# Autodesk Inventor assembly: Tiger
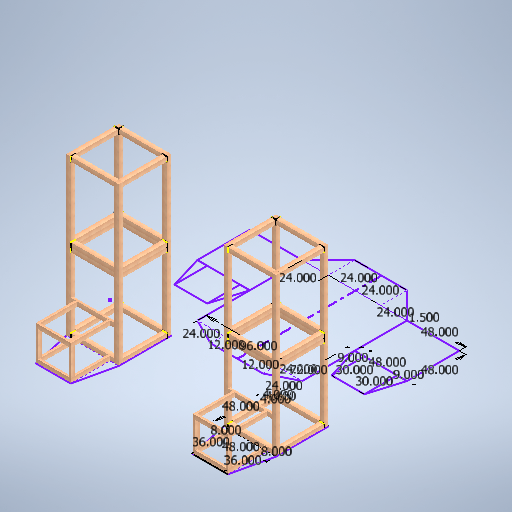
[picture p0: Inventor's stored thumbnail of the model, 512x512]
Saved by Autodesk Inventor 2025 (Build 290162000, 162)
## iProperties
Created: 2024-06-05
Part Number: Tiger
Document SubType Name: Assembly
Designer: Cupri
Mass: 180546 g
Surface Area: 136258 cm^2
Volume: 328266 cm^3
Density: 0.55 g/cm^3
Author: Cupri
## Documents named in this file (13)
- C:\Users\Cupri\OneDrive\Documents\TigerBurn\USCTigerBurn24\v1\Tiger.iam
- C:\Users\Cupri\OneDrive\Documents\TigerBurn\USCTigerBurn24\Standard Timber\4x4x72.ipt
- C:\Users\Cupri\OneDrive\Documents\TigerBurn\USCTigerBurn24\Standard Timber\4x4x40.ipt
- C:\Users\Cupri\OneDrive\Documents\TigerBurn\USCTigerBurn24\Standard Timber\2x4x36.ipt
- C:\Users\Cupri\OneDrive\Documents\TigerBurn\USCTigerBurn24\Standard Timber\2x4x40.ipt
- C:\Users\Cupri\OneDrive\Documents\TigerBurn\USCTigerBurn24\Standard Timber\2x4x24.ipt
- C:\Users\Cupri\OneDrive\Documents\TigerBurn\USCTigerBurn24\Standard Timber\2x4x28.ipt
- C:\Users\Cupri\OneDrive\Documents\TigerBurn\USCTigerBurn24\v1\Tiger\AIP\FEA\epzzwi8io.fins
- C:\Users\Cupri\OneDrive\Documents\TigerBurn\USCTigerBurn24\v1\Tiger\AIP\FEA\epzzwi8io.fsat
- C:\Users\Cupri\OneDrive\Documents\TigerBurn\USCTigerBurn24\v1\Tiger\AIP\FEA\epzzwi8io.ftes
- C:\Users\Cupri\OneDrive\Documents\TigerBurn\USCTigerBurn24\v1\Tiger\AIP\FEA\epzzwi8io.fwiz
- C:\Users\Cupri\OneDrive\Documents\TigerBurn\USCTigerBurn24\v1\Tiger\AIP\FEA\epzzwi8jk.fmsh
- C:\Users\Cupri\OneDrive\Documents\TigerBurn\USCTigerBurn24\v1\Tiger\AIP\FEA\epzzwi8jl.fres
## Components (66 placed, 6 different names)
1. 4x4x72:9
2. 4x4x72:10
3. 4x4x40:17 — Flush:14
4. 4x4x40:18
5. 4x4x40:19 — Mate:19, Mate:20
6. 4x4x40:20 — Flush:13, Mate:18
7. 4x4x40:21
8. 4x4x40:22
9. 4x4x40:23
10. 4x4x40:24
11. 4x4x72:11
12. 4x4x72:12 — Mate:21
13. 4x4x72:13
14. 4x4x72:14
15. 4x4x40:25
16. 4x4x40:26
17. 4x4x40:27
18. 4x4x40:28
19. 4x4x40:29
20. 4x4x40:30
21. 4x4x40:31
22. 4x4x40:32
23. 4x4x72:15
24. 4x4x72:16
25. 2x4x40:2 — Mate:21, Mate:23
26. 2x4x36:5 — Mate:20
27. 2x4x36:6 — Mate:23, Mate:24
28. 2x4x36:7 — Mate:22
29. 2x4x36:8 — Mate:19
30. 2x4x24:3
31. 2x4x24:4 — Mate:22
32. 2x4x28:3 — Mate:24
33. 2x4x28:4
34. 4x4x72:1 — Rigid:1, Rigid:3, Rigid:10, Rigid:11
35. 4x4x72:2 — Rigid:2, Rigid:4, Rigid:8
36. 4x4x40:1 — Rigid:1, Rigid:2, Flush:14
37. 4x4x40:2 — Rigid:3, Rigid:5, Flush:13, Mate:18
38. 4x4x40:3 — Rigid:6, Mate:5, Mate:6, Flush:4, Flush:5
39. 4x4x40:4 — Rigid:4, Rigid:7
40. 4x4x40:5 — Rigid:8
41. 4x4x40:6 — Rigid:9, Rigid:23
42. 4x4x40:7 — Rigid:11
43. 4x4x40:8 — Rigid:10
44. 4x4x72:3 — Rigid:5, Rigid:6, Rigid:9, Mate:4, Flush:3
45. 4x4x72:4 — Rigid:7, Mate:7
46. 4x4x72:5
47. 4x4x72:6
48. 4x4x40:9
49. 4x4x40:10
50. 4x4x40:11 — Rigid:23
51. 4x4x40:12
52. 4x4x40:13
53. 4x4x40:14
54. 4x4x40:15
55. 4x4x40:16
56. 4x4x72:7
57. 4x4x72:8
58. 2x4x40:1 — Mate:4, Flush:3, Mate:5, Mate:8, Flush:6, Mate:9, Flush:7
59. 2x4x36:1 — Mate:6, Flush:4, Rigid:24
60. 2x4x36:2 — Mate:8, Flush:6
61. 2x4x36:3 — Mate:9, Flush:7, Mate:10, Rigid:26
62. 2x4x36:4 — Mate:7, Flush:5, Mate:10, Rigid:25, Rigid:27
63. 2x4x24:1 — Rigid:24
64. 2x4x24:2 — Rigid:25
65. 2x4x28:1 — Rigid:26
66. 2x4x28:2 — Rigid:27
## Relationships (86: WeldJoint 54, Mate 20, Flush 12)
- Rigid:1 [WeldJoint]: 4x4x72:1 ↔ 4x4x40:1
- Rigid:2 [WeldJoint]: 4x4x72:2 ↔ 4x4x40:1
- Rigid:3 [WeldJoint]: 4x4x72:1 ↔ 4x4x40:2
- Rigid:4 [WeldJoint]: 4x4x72:2 ↔ 4x4x40:4
- Rigid:5 [WeldJoint]: 4x4x40:2 ↔ 4x4x72:3
- Rigid:6 [WeldJoint]: 4x4x40:3 ↔ 4x4x72:3
- Rigid:7 [WeldJoint]: 4x4x40:4 ↔ 4x4x72:4
- Rigid:8 [WeldJoint]: 4x4x72:2 ↔ 4x4x40:5
- Rigid:9 [WeldJoint]: 4x4x40:6 ↔ 4x4x72:3
- Rigid:10 [WeldJoint]: 4x4x72:1 ↔ 4x4x40:8
- Rigid:11 [WeldJoint]: 4x4x72:1 ↔ 4x4x40:7
- [WeldJoint]: 4x4x72:5 ↔ 4x4x40:9
- [WeldJoint]: 4x4x72:6 ↔ 4x4x40:9
- [WeldJoint]: 4x4x72:5 ↔ 4x4x40:10
- [WeldJoint]: 4x4x72:6 ↔ 4x4x40:12
- [WeldJoint]: 4x4x40:10 ↔ 4x4x72:7
- [WeldJoint]: 4x4x40:11 ↔ 4x4x72:7
- [WeldJoint]: 4x4x40:12 ↔ 4x4x72:8
- [WeldJoint]: 4x4x72:6 ↔ 4x4x40:13
- [WeldJoint]: 4x4x40:14 ↔ 4x4x72:7
- [WeldJoint]: 4x4x72:5 ↔ 4x4x40:16
- [WeldJoint]: 4x4x72:5 ↔ 4x4x40:15
- Rigid:23 [WeldJoint]: 4x4x40:6 ↔ 4x4x40:11
- Mate:4: 4x4x72:3 ↔ 2x4x40:1
- Flush:3: 4x4x72:3 ↔ 2x4x40:1
- Mate:5 (609.6 mm): 4x4x40:3 ↔ 2x4x40:1
- Mate:6 (101.6 mm): 4x4x40:3 ↔ 2x4x36:1
- Flush:4: 4x4x40:3 ↔ 2x4x36:1
- Mate:7 (101.6 mm): 4x4x72:4 ↔ 2x4x36:4
- Flush:5: 4x4x40:3 ↔ 2x4x36:4
- Mate:8 (101.6 mm): 2x4x40:1 ↔ 2x4x36:2
- Flush:6: 2x4x40:1 ↔ 2x4x36:2
- Mate:9: 2x4x40:1 ↔ 2x4x36:3
- Flush:7: 2x4x40:1 ↔ 2x4x36:3
- Mate:10: 2x4x36:3 ↔ 2x4x36:4
- Rigid:24 [WeldJoint]: 2x4x36:1 ↔ 2x4x24:1
- Rigid:25 [WeldJoint]: 2x4x36:4 ↔ 2x4x24:2
- Rigid:26 [WeldJoint]: 2x4x36:3 ↔ 2x4x28:1
- Rigid:27 [WeldJoint]: 2x4x36:4 ↔ 2x4x28:2
- [WeldJoint]: 4x4x72:9 ↔ 4x4x40:17
- [WeldJoint]: 4x4x72:10 ↔ 4x4x40:17
- [WeldJoint]: 4x4x72:9 ↔ 4x4x40:18
- [WeldJoint]: 4x4x72:10 ↔ 4x4x40:20
- [WeldJoint]: 4x4x40:18 ↔ 4x4x72:11
- [WeldJoint]: 4x4x40:19 ↔ 4x4x72:11
- [WeldJoint]: 4x4x40:20 ↔ 4x4x72:12
- [WeldJoint]: 4x4x72:10 ↔ 4x4x40:21
- [WeldJoint]: 4x4x40:22 ↔ 4x4x72:11
- [WeldJoint]: 4x4x72:9 ↔ 4x4x40:24
- [WeldJoint]: 4x4x72:9 ↔ 4x4x40:23
- [WeldJoint]: 4x4x72:13 ↔ 4x4x40:25
- [WeldJoint]: 4x4x72:14 ↔ 4x4x40:25
- [WeldJoint]: 4x4x72:13 ↔ 4x4x40:26
- [WeldJoint]: 4x4x72:14 ↔ 4x4x40:28
- [WeldJoint]: 4x4x40:26 ↔ 4x4x72:15
- [WeldJoint]: 4x4x40:27 ↔ 4x4x72:15
- [WeldJoint]: 4x4x40:28 ↔ 4x4x72:16
- [WeldJoint]: 4x4x72:14 ↔ 4x4x40:29
- [WeldJoint]: 4x4x40:30 ↔ 4x4x72:15
- [WeldJoint]: 4x4x72:13 ↔ 4x4x40:32
- [WeldJoint]: 4x4x72:13 ↔ 4x4x40:31
- [WeldJoint]: 4x4x40:22 ↔ 4x4x40:27
- [Mate]: 4x4x72:11 ↔ 2x4x40:2
- [Flush]: 4x4x72:11 ↔ 2x4x40:2
- [Mate] (609.6 mm): 4x4x40:19 ↔ 2x4x40:2
- [Mate] (101.6 mm): 4x4x40:19 ↔ 2x4x36:5
- [Flush]: 4x4x40:19 ↔ 2x4x36:5
- [Mate] (101.6 mm): 4x4x72:12 ↔ 2x4x36:8
- [Flush]: 4x4x40:19 ↔ 2x4x36:8
- [Flush]: 2x4x40:2 ↔ 2x4x36:6
- [Mate]: 2x4x40:2 ↔ 2x4x36:7
- [Flush]: 2x4x40:2 ↔ 2x4x36:7
- [Mate]: 2x4x36:7 ↔ 2x4x36:8
- [WeldJoint]: 2x4x36:5 ↔ 2x4x24:3
- [WeldJoint]: 2x4x36:8 ↔ 2x4x24:4
- [WeldJoint]: 2x4x36:7 ↔ 2x4x28:3
- [WeldJoint]: 2x4x36:8 ↔ 2x4x28:4
- Flush:13: 4x4x40:20 ↔ 4x4x40:2
- Mate:18 (2438.4 mm): 4x4x40:20 ↔ 4x4x40:2
- Flush:14: 4x4x40:17 ↔ 4x4x40:1
- Mate:19: 4x4x40:19 ↔ 2x4x36:8
- Mate:20: 4x4x40:19 ↔ 2x4x36:5
- Mate:21: 4x4x72:12 ↔ 2x4x40:2
- Mate:22: 2x4x36:7 ↔ 2x4x24:4
- Mate:23: 2x4x40:2 ↔ 2x4x36:6
- Mate:24: 2x4x36:6 ↔ 2x4x28:3
## Named parameters: d40_d29 = 0 mm, d41_d30 = 0 mm, d42_d31 = 0 mm, d43_d32 = 0 mm, d44_d33 = 0 mm, d45_d34 = 0 mm, d46_d35 = 0 mm, d47_d36 = 0 mm, d48_d37 = 0 mm, d49_d38 = 0 mm, d50_d39 = 0 mm, sa_0 = 22241.1, d81_d51 = 0 mm, d82_d31 = 0 mm, d83_d32 = 0 mm, d84_d33 = 0 mm, d85_d34 = 0 mm, d86_d35 = 0 mm, d87_d36 = 0 mm, d88_d37 = 0 mm, d89_d38 = 0 mm, d90_d39 = 0 mm, d91_d40_d29 = 0 mm, d92_d41_d30 = 0 mm, d93_d42_d31 = 0 mm, d94_d43_d32 = 0 mm, d95_d44_d33 = 0 mm, d96_d45_d34 = 0 mm, d97_d46_d35 = 0 mm, d98_d47_d36 = 0 mm, d99_d48_d37 = 0 mm, d100_d49_d38 = 0 mm, d101_d50_d39 = 0 mm, d102_d29 = 0 mm, d103_d30 = 0 mm, d104_d75 = 0 mm, d105_d76 = 0 mm, d106_d77 = 0 mm, d107_d78 = 0 mm, d108_d79 = 0 mm, d109_d80 = 0 mm, d110_d68 = 101.6 mm, d111_d69 = 0 mm, d112_d70 = 101.6 mm, d113_d71 = 0 mm, d115_d73 = 0 mm, d116_d74 = 0 mm, d117_d61 = 0 mm, d118_d62 = 0 mm, d119_d63 = 609.6 mm
note: some values were not read from the file. Shown as the stored number, unit unknown: "sa_0".
